# Autodesk Inventor assembly: POM_T5_10
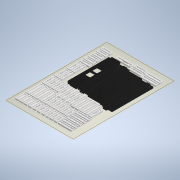
[picture p0: Inventor's stored thumbnail of the model, 180x180]
Saved by Autodesk Inventor 2020 (Build 240168000, 168)
## iProperties
Created: 2021-08-27
Part Number: POM_T5_10
Document SubType Name: Assembly
Designer: Masato
Author: Masato
## Documents named in this file (16)
- D:\GitHub\inventor\SUSTAINA-OP\Cam\POM_T5_10.iam
- D:\GitHub\inventor\SUSTAINA-OP\Cam\DisposableBoard.ipt
- D:\GitHub\inventor\SUSTAINA-OP\Jig\BackLink_diagonal_Jig.ipt
- D:\GitHub\inventor\SUSTAINA-OP\Jig\Foot_root_block_Jig.ipt
- D:\GitHub\inventor\SUSTAINA-OP\Jig\FrontLink_diagonal_Jig.ipt
- D:\GitHub\inventor\SUSTAINA-OP\Jig\Head_horn_frame_Jig.ipt
- D:\GitHub\inventor\SUSTAINA-OP\Jig\Leg_joint_yaw_frame_Jig.ipt
- D:\GitHub\inventor\SUSTAINA-OP\Jig\Shoulder_horn_frame_Jig.ipt
- D:\GitHub\inventor\SUSTAINA-OP\Jig\Trunk_chest_frame_Jig_1.ipt
- D:\GitHub\inventor\SUSTAINA-OP\Jig\Trunk_lower_side_frame_Jig.ipt
- D:\GitHub\inventor\SUSTAINA-OP\Jig\Trunk_chest_frame_Jig_2.ipt
- D:\GitHub\inventor\SUSTAINA-OP\Jig\UpperArm_diagonal_Jig.ipt
- D:\GitHub\inventor\SUSTAINA-OP\UpperBody\Cockpit\Cockpit_battery_bottom_frame.ipt
- D:\GitHub\inventor\SUSTAINA-OP\UpperBody\Cockpit\Cockpit_battery_back_door.ipt
- D:\GitHub\inventor\SUSTAINA-OP\UpperBody\Cockpit\Cockpit_battery_front_frame.ipt
- D:\GitHub\inventor\SUSTAINA-OP\UpperBody\Cockpit\Cockpit_top_frame.ipt
## Components (58 placed, 15 different names)
1. DisposableBoard:1 — メイト:2, メイト:1, フラッシュ:1, フラッシュ:2, メイト:4, メイト:5, メイト:6, メイト:10, メイト:11, メイト:13, メイト:15, メイト:17, メイト:20, メイト:21, メイト:23, メイト:25, メイト:26, メイト:28, メイト:29, メイト:32, メイト:35, メイト:43, メイト:46, メイト:47, メイト:48, メイト:49, メイト:50, メイト:58, メイト:60, メイト:62, メイト:63, メイト:65, メイト:66, メイト:68, メイト:69, メイト:70, メイト:73, メイト:76
2. UpperArm_diagonal_Jig:4 — メイト:43, メイト:44, メイト:45
3. Cockpit_battery_back_door:1 — メイト:47, メイト:52, メイト:53, メイト:54
4. Cockpit_battery_bottom_frame:1 — メイト:46, メイト:50, メイト:52, メイト:71, メイト:72
5. Cockpit_battery_front_frame:1 — メイト:48, メイト:54, メイト:55, メイト:56, メイト:75
6. Cockpit_top_frame:1 — メイト:49, メイト:56, メイト:57, メイト:78
7. Trunk_chest_frame_Jig_2:5 — メイト:76, メイト:77, メイト:78
8. BackLink_diagonal_Jig:2 — メイト:4, メイト:5, メイト:6, メイト:14
9. BackLink_diagonal_Jig:3
10. BackLink_diagonal_Jig:4
11. BackLink_diagonal_Jig:5 — メイト:16
12. Foot_root_block_Jig:1 — メイト:10, メイト:11, メイト:16, メイト:18
13. Foot_root_block_Jig:2
14. Foot_root_block_Jig:3
15. Foot_root_block_Jig:4 — メイト:22
16. FrontLink_diagonal_Jig:1 — メイト:13, メイト:14, メイト:15, メイト:27
17. FrontLink_diagonal_Jig:2
18. FrontLink_diagonal_Jig:3
19. FrontLink_diagonal_Jig:4 — メイト:19
20. Head_horn_frame_Jig:1 — メイト:17, メイト:18, メイト:19, メイト:30
21. Head_horn_frame_Jig:2
22. Head_horn_frame_Jig:3
23. Head_horn_frame_Jig:4
24. Trunk_chest_frame_Jig_1:2 — メイト:23, メイト:24, メイト:25
25. Trunk_chest_frame_Jig_1:3
26. Trunk_chest_frame_Jig_1:4
27. Trunk_chest_frame_Jig_1:5
28. Trunk_chest_frame_Jig_1:6 — メイト:33, メイト:45
29. Shoulder_horn_frame_Jig:1 — メイト:26, メイト:27, メイト:28, メイト:59
30. Shoulder_horn_frame_Jig:2
31. Shoulder_horn_frame_Jig:3
32. Shoulder_horn_frame_Jig:4 — メイト:31, メイト:57
33. Trunk_lower_side_frame_Jig:1 — メイト:29, メイト:30, メイト:31
34. Trunk_lower_side_frame_Jig:2
35. Trunk_lower_side_frame_Jig:3 — メイト:55
36. Trunk_lower_side_frame_Jig:4 — メイト:34, メイト:53
37. Trunk_chest_frame_Jig_2:1 — メイト:32, メイト:33, メイト:34
38. Trunk_chest_frame_Jig_2:2
39. Trunk_chest_frame_Jig_2:3
40. Trunk_chest_frame_Jig_2:4 — メイト:44, メイト:72
41. UpperArm_diagonal_Jig:1 — メイト:35, メイト:58, メイト:59
42. UpperArm_diagonal_Jig:5
43. UpperArm_diagonal_Jig:6
44. UpperArm_diagonal_Jig:7 — メイト:61
45. BackLink_diagonal_Jig:6 — メイト:60, メイト:61, メイト:62
46. BackLink_diagonal_Jig:7 — メイト:64
47. Foot_root_block_Jig:5 — メイト:63, メイト:64, メイト:65
48. Foot_root_block_Jig:6 — メイト:67
49. Leg_joint_yaw_frame_Jig:5 — メイト:66, メイト:67, メイト:68
50. Leg_joint_yaw_frame_Jig:6
51. FrontLink_diagonal_Jig:5 — メイト:69, メイト:70, メイト:71, メイト:74
52. FrontLink_diagonal_Jig:6
53. Head_horn_frame_Jig:5 — メイト:73, メイト:74, メイト:75
54. Head_horn_frame_Jig:6 — メイト:77
55. Leg_joint_yaw_frame_Jig:1 — メイト:20, メイト:21, メイト:22
56. Leg_joint_yaw_frame_Jig:2 — メイト:24
57. Leg_joint_yaw_frame_Jig:3
58. Leg_joint_yaw_frame_Jig:4
## Component patterns: (4 elements, first: BackLink_diagonal_Jig:2), (4 elements, first: Foot_root_block_Jig:1), (4 elements, first: FrontLink_diagonal_Jig:1), (4 elements, first: Head_horn_frame_Jig:1), (2 elements), (5 elements, first: Trunk_chest_frame_Jig_1:2), (4 elements, first: Shoulder_horn_frame_Jig:1), (4 elements, first: Trunk_lower_side_frame_Jig:1), (4 elements, first: Trunk_chest_frame_Jig_2:1), (4 elements, first: UpperArm_diagonal_Jig:1), (2 elements, first: BackLink_diagonal_Jig:6), (2 elements, first: Foot_root_block_Jig:5), (2 elements, first: Leg_joint_yaw_frame_Jig:5), (2 elements, first: FrontLink_diagonal_Jig:5), (2 elements, first: Head_horn_frame_Jig:5), (2 elements, first: Leg_joint_yaw_frame_Jig:1), コンポーネント パターン 6:2 (2 elements)
## Relationships (67: Mate 65, Flush 2)
- メイト:2 [Mate]: DisposableBoard:1
- メイト:1 [Mate]: DisposableBoard:1
- フラッシュ:1 [Flush]: DisposableBoard:1
- フラッシュ:2 [Flush]: DisposableBoard:1
- メイト:4 [Mate]: DisposableBoard:1 ↔ BackLink_diagonal_Jig:2
- メイト:5 [Mate] (2.5 mm): DisposableBoard:1 ↔ BackLink_diagonal_Jig:2
- メイト:6 [Mate] (2.5 mm): DisposableBoard:1 ↔ BackLink_diagonal_Jig:2
- メイト:10 [Mate]: DisposableBoard:1 ↔ Foot_root_block_Jig:1
- メイト:11 [Mate] (2.5 mm): DisposableBoard:1 ↔ Foot_root_block_Jig:1
- メイト:13 [Mate]: DisposableBoard:1 ↔ FrontLink_diagonal_Jig:1
- メイト:14 [Mate] (3 mm): BackLink_diagonal_Jig:2 ↔ FrontLink_diagonal_Jig:1
- メイト:15 [Mate] (2.5 mm): DisposableBoard:1 ↔ FrontLink_diagonal_Jig:1
- メイト:16 [Mate] (3 mm): BackLink_diagonal_Jig:5 ↔ Foot_root_block_Jig:1
- メイト:17 [Mate]: DisposableBoard:1 ↔ Head_horn_frame_Jig:1
- メイト:18 [Mate] (3 mm): Foot_root_block_Jig:1 ↔ Head_horn_frame_Jig:1
- メイト:19 [Mate] (3 mm): FrontLink_diagonal_Jig:4 ↔ Head_horn_frame_Jig:1
- メイト:20 [Mate]: DisposableBoard:1 ↔ Leg_joint_yaw_frame_Jig:1
- メイト:21 [Mate] (2.5 mm): DisposableBoard:1 ↔ Leg_joint_yaw_frame_Jig:1
- メイト:22 [Mate] (3 mm): Foot_root_block_Jig:4 ↔ Leg_joint_yaw_frame_Jig:1
- メイト:23 [Mate]: DisposableBoard:1 ↔ Trunk_chest_frame_Jig_1:2
- メイト:24 [Mate] (3 mm): Trunk_chest_frame_Jig_1:2 ↔ Leg_joint_yaw_frame_Jig:2
- メイト:25 [Mate] (2.5 mm): DisposableBoard:1 ↔ Trunk_chest_frame_Jig_1:2
- メイト:26 [Mate]: DisposableBoard:1 ↔ Shoulder_horn_frame_Jig:1
- メイト:27 [Mate] (3 mm): FrontLink_diagonal_Jig:1 ↔ Shoulder_horn_frame_Jig:1
- メイト:28 [Mate] (2.5 mm): DisposableBoard:1 ↔ Shoulder_horn_frame_Jig:1
- メイト:29 [Mate]: DisposableBoard:1 ↔ Trunk_lower_side_frame_Jig:1
- メイト:30 [Mate] (3 mm): Head_horn_frame_Jig:1 ↔ Trunk_lower_side_frame_Jig:1
- メイト:31 [Mate] (3 mm): Shoulder_horn_frame_Jig:4 ↔ Trunk_lower_side_frame_Jig:1
- メイト:32 [Mate]: DisposableBoard:1 ↔ Trunk_chest_frame_Jig_2:1
- メイト:33 [Mate] (3 mm): Trunk_chest_frame_Jig_1:6 ↔ Trunk_chest_frame_Jig_2:1
- メイト:34 [Mate] (3 mm): Trunk_lower_side_frame_Jig:4 ↔ Trunk_chest_frame_Jig_2:1
- メイト:35 [Mate]: DisposableBoard:1 ↔ UpperArm_diagonal_Jig:1
- メイト:43 [Mate]: DisposableBoard:1 ↔ UpperArm_diagonal_Jig:4
- メイト:44 [Mate] (3 mm): UpperArm_diagonal_Jig:4 ↔ Trunk_chest_frame_Jig_2:4
- メイト:45 [Mate] (3 mm): UpperArm_diagonal_Jig:4 ↔ Trunk_chest_frame_Jig_1:6
- メイト:46 [Mate]: DisposableBoard:1 ↔ Cockpit_battery_bottom_frame:1
- メイト:47 [Mate]: DisposableBoard:1 ↔ Cockpit_battery_back_door:1
- メイト:48 [Mate]: DisposableBoard:1 ↔ Cockpit_battery_front_frame:1
- メイト:49 [Mate]: DisposableBoard:1 ↔ Cockpit_top_frame:1
- メイト:50 [Mate] (3 mm): DisposableBoard:1 ↔ Cockpit_battery_bottom_frame:1
- メイト:52 [Mate] (2.5 mm): Cockpit_battery_back_door:1 ↔ Cockpit_battery_bottom_frame:1
- メイト:53 [Mate] (4 mm): Cockpit_battery_back_door:1 ↔ Trunk_lower_side_frame_Jig:4
- メイト:54 [Mate] (2.5 mm): Cockpit_battery_back_door:1 ↔ Cockpit_battery_front_frame:1
- メイト:55 [Mate] (3 mm): Cockpit_battery_front_frame:1 ↔ Trunk_lower_side_frame_Jig:3
- メイト:56 [Mate] (2.5 mm): Cockpit_battery_front_frame:1 ↔ Cockpit_top_frame:1
- メイト:57 [Mate] (3 mm): Cockpit_top_frame:1 ↔ Shoulder_horn_frame_Jig:4
- メイト:58 [Mate] (2.5 mm): DisposableBoard:1 ↔ UpperArm_diagonal_Jig:1
- メイト:59 [Mate] (2.5 mm): Shoulder_horn_frame_Jig:1 ↔ UpperArm_diagonal_Jig:1
- メイト:60 [Mate]: DisposableBoard:1 ↔ BackLink_diagonal_Jig:6
- メイト:61 [Mate] (2.5 mm): UpperArm_diagonal_Jig:7 ↔ BackLink_diagonal_Jig:6
- メイト:62 [Mate] (2.5 mm): DisposableBoard:1 ↔ BackLink_diagonal_Jig:6
- メイト:63 [Mate]: DisposableBoard:1 ↔ Foot_root_block_Jig:5
- メイト:64 [Mate] (2.5 mm): BackLink_diagonal_Jig:7 ↔ Foot_root_block_Jig:5
- メイト:65 [Mate] (2.5 mm): DisposableBoard:1 ↔ Foot_root_block_Jig:5
- メイト:66 [Mate]: DisposableBoard:1 ↔ Leg_joint_yaw_frame_Jig:5
- メイト:67 [Mate] (2.5 mm): Foot_root_block_Jig:6 ↔ Leg_joint_yaw_frame_Jig:5
- メイト:68 [Mate] (2.5 mm): DisposableBoard:1 ↔ Leg_joint_yaw_frame_Jig:5
- メイト:69 [Mate]: DisposableBoard:1 ↔ FrontLink_diagonal_Jig:5
- メイト:70 [Mate] (2.5 mm): DisposableBoard:1 ↔ FrontLink_diagonal_Jig:5
- メイト:71 [Mate] (2.5 mm): Cockpit_battery_bottom_frame:1 ↔ FrontLink_diagonal_Jig:5
- メイト:72 [Mate] (2.5 mm): Cockpit_battery_bottom_frame:1 ↔ Trunk_chest_frame_Jig_2:4
- メイト:73 [Mate]: DisposableBoard:1 ↔ Head_horn_frame_Jig:5
- メイト:74 [Mate] (2.5 mm): FrontLink_diagonal_Jig:5 ↔ Head_horn_frame_Jig:5
- メイト:75 [Mate] (2.5 mm): Cockpit_battery_front_frame:1 ↔ Head_horn_frame_Jig:5
- メイト:76 [Mate]: DisposableBoard:1 ↔ Trunk_chest_frame_Jig_2:5
- メイト:77 [Mate] (2.5 mm): Trunk_chest_frame_Jig_2:5 ↔ Head_horn_frame_Jig:6
- メイト:78 [Mate] (2.5 mm): Cockpit_top_frame:1 ↔ Trunk_chest_frame_Jig_2:5
